# Autodesk Inventor assembly: balljoint_asm
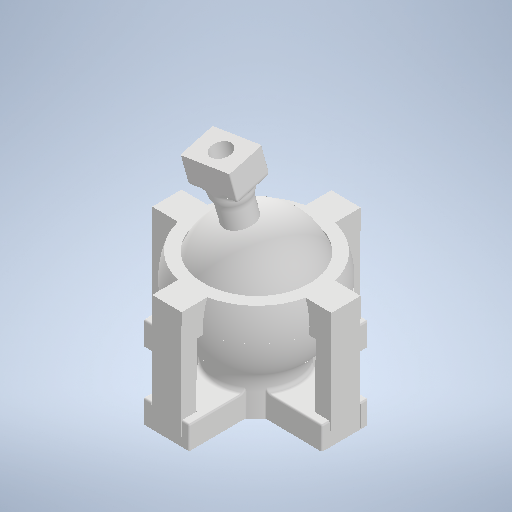
[picture p0: Inventor's stored thumbnail of the model, 512x512]
Saved by Autodesk Inventor 2025.1 (Build 291241000, 241)
## iProperties
Created: 2024-11-01
Part Number: balljoint_asm
Document SubType Name: Assembly
Designer: ZOMBULLI
Author: ZOMBULLI
## Documents named in this file (4)
- C:\Users\xingj\Downloads\CAD\Stewart Platform_new\balljoint_asm.iam
- C:\Users\xingj\Downloads\CAD\Stewart Platform_new\female_1,3.ipt
- C:\Users\xingj\Downloads\CAD\Stewart Platform_new\clip_1,3.ipt
- C:\Users\xingj\Downloads\CAD\Stewart Platform_new\balljoint_male.ipt
## Components (3 placed, 3 different names)
1. female_1,3:1 — Mate:1, Mate:2, Mate:3, Tangent:1, Mate:4
2. clip_1,3:1 — Mate:1, Mate:2, Mate:3, Mate:4, Mate:5
3. balljoint_male:1 — Tangent:1, Mate:5
## Relationships (6: Mate 5, Tangent 1)
- Mate:1: female_1,3:1 ↔ clip_1,3:1
- Mate:2: female_1,3:1 ↔ clip_1,3:1
- Mate:3: female_1,3:1 ↔ clip_1,3:1
- Tangent:1: female_1,3:1 ↔ balljoint_male:1
- Mate:4: female_1,3:1 ↔ clip_1,3:1
- Mate:5: clip_1,3:1 ↔ balljoint_male:1
